# Autodesk Inventor assembly: cover assembly
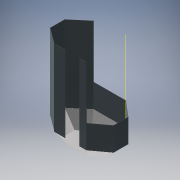
[picture p0: Inventor's stored thumbnail of the model, 180x180]
Saved by Autodesk Inventor 2016 (Build 200138000, 138)
## iProperties
Created: 2017-08-22
Part Number: cover assembly
Document SubType Name: Assembly
Designer: m227586
Author: m227586
## Documents named in this file (3)
- E:\Lathe with updated parts (LATEST of 20 06 17)\cover parts\cover assembly.iam
- E:\Lathe with updated parts (LATEST of 20 06 17)\cover parts\Cover end.ipt
- E:\Lathe with updated parts (LATEST of 20 06 17)\cover parts\Main Cover.ipt
## Components (2 placed, 2 different names)
1. Cover end:1 — Mate:6, Mate:8, Mate:9
2. Main Cover:1 — Mate:6, Mate:7, Mate:8, Mate:9
## Relationships (4: Mate 4)
- Mate:6: Cover end:1 ↔ Main Cover:1
- Mate:7: Main Cover:1
- Mate:8: Cover end:1 ↔ Main Cover:1
- Mate:9: Cover end:1 ↔ Main Cover:1
